# Autodesk Inventor assembly: Montagem3
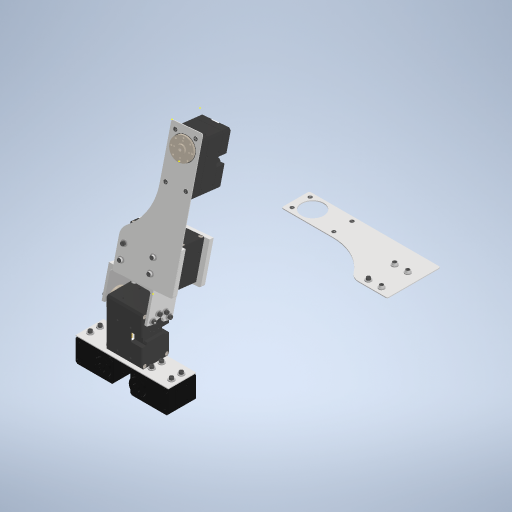
[picture p0: Inventor's stored thumbnail of the model, 512x512]
Saved by Autodesk Inventor 2024 (Build 280153000, 153)
## iProperties
Created: 2024-10-14
Part Number: Montagem3
Document SubType Name: Assembly
Designer: robof
Author: robof
## Documents named in this file (7)
- C:\Github_mecanica\Artigo\componentes\Montagem3.iam
- C:\Github_mecanica\Artigo\componentes\Dynamixel_XM540.ipt
- C:\Github_mecanica\Artigo\componentes\linkzinho_motor.ipt
- C:\Github_mecanica\Artigo\componentes\chapinha_garra.ipt
- C:\Github_mecanica\Artigo\componentes\XM430-W350-R.ipt
- C:\Github_mecanica\Artigo\componentes\chapa_carbono_lateral.ipt
- C:\Github_mecanica\Artigo\componentes\Calco.ipt
## Components (11 placed, 6 different names)
1. chapinha_garra:1 — Alinhado:1, Coincidente:1, Coincidente:2, Coincidente:3, Alinhado:2, Alinhado:3, Coincidente:4, Alinhado:4, Alinhado:5, Coincidente:5, Coincidente:6, Coincidente:7
2. XM430-W350-R:1 — Coincidente:4, Alinhado:4, Alinhado:5
3. XM430-W350-R:2 — Coincidente:3, Alinhado:2, Alinhado:3
4. Dynamixel_XM540:1 — Coincidente:5, Coincidente:6, Coincidente:7, Coincidente:8, Coincidente:9
5. linkzinho_motor:1 — Coincidente:8, Coincidente:9, Coincidente:10, Coincidente:11, Coincidente:20
6. Dynamixel_XM540:2 — Coincidente:10, Coincidente:11, Coincidente:12, Coincidente:13, Coincidente:14, Coincidente:15, Coincidente:16
7. chapa_carbono_lateral:2 — Coincidente:18, Coincidente:19, Coincidente:20, Coincidente:21
8. Calco:1 — Coincidente:15, Coincidente:16, Coincidente:17
9. Calco:2 — Coincidente:12, Coincidente:13, Coincidente:14, Coincidente:17, Coincidente:18, Coincidente:19
10. chapa_carbono_lateral:3
11. Dynamixel_XM540:3 — Coincidente:21
## Relationships (26: Mate 21, Flush 5)
- Alinhado:1 [Flush]: chapinha_garra:1
- Coincidente:1 [Mate]: chapinha_garra:1
- Coincidente:2 [Mate]: chapinha_garra:1
- Coincidente:3 [Mate]: chapinha_garra:1 ↔ XM430-W350-R:2
- Alinhado:2 [Flush]: chapinha_garra:1 ↔ XM430-W350-R:2
- Alinhado:3 [Flush]: chapinha_garra:1 ↔ XM430-W350-R:2
- Coincidente:4 [Mate]: chapinha_garra:1 ↔ XM430-W350-R:1
- Alinhado:4 [Flush]: chapinha_garra:1 ↔ XM430-W350-R:1
- Alinhado:5 [Flush]: chapinha_garra:1 ↔ XM430-W350-R:1
- Coincidente:5 [Mate]: chapinha_garra:1 ↔ Dynamixel_XM540:1
- Coincidente:6 [Mate]: chapinha_garra:1 ↔ Dynamixel_XM540:1
- Coincidente:7 [Mate] (34.5 mm): chapinha_garra:1 ↔ Dynamixel_XM540:1
- Coincidente:8 [Mate]: Dynamixel_XM540:1 ↔ linkzinho_motor:1
- Coincidente:9 [Mate]: Dynamixel_XM540:1 ↔ linkzinho_motor:1
- Coincidente:10 [Mate]: linkzinho_motor:1 ↔ Dynamixel_XM540:2
- Coincidente:11 [Mate]: linkzinho_motor:1 ↔ Dynamixel_XM540:2
- Coincidente:12 [Mate]: Dynamixel_XM540:2 ↔ Calco:2
- Coincidente:13 [Mate]: Dynamixel_XM540:2 ↔ Calco:2
- Coincidente:14 [Mate] (5.5 mm): Dynamixel_XM540:2 ↔ Calco:2
- Coincidente:15 [Mate]: Dynamixel_XM540:2 ↔ Calco:1
- Coincidente:16 [Mate]: Dynamixel_XM540:2 ↔ Calco:1
- Coincidente:17 [Mate] (33.52 mm): Calco:1 ↔ Calco:2
- Coincidente:18 [Mate]: chapa_carbono_lateral:2 ↔ Calco:2
- Coincidente:19 [Mate]: chapa_carbono_lateral:2 ↔ Calco:2
- Coincidente:20 [Mate]: linkzinho_motor:1 ↔ chapa_carbono_lateral:2
- Coincidente:21 [Mate]: chapa_carbono_lateral:2 ↔ Dynamixel_XM540:3
